# Autodesk Inventor assembly: Assembly
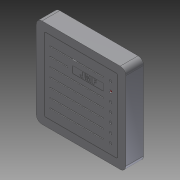
[picture p0: Inventor's stored thumbnail of the model, 180x180]
Saved by Autodesk Inventor 2012 (Build 160160000, 160)
## iProperties
Created: 2013-12-16
Part Number: Assembly
Document SubType Name: Assembly
Designer: joe_000
Author: joe_000
## Documents named in this file (5)
- C:\dev\stm32-rfid-clone\mechanical\Assembly.iam
- C:\dev\stm32-rfid-clone\mechanical\readerCase.ipt
- C:\dev\stm32-rfid-clone\mechanical\AABattery.ipt
- C:\dev\stm32-rfid-clone\mechanical\circuitBoard.ipt
- C:\dev\stm32-rfid-clone\mechanical\LED.ipt
## Components (7 placed, 4 different names)
1. readerCase:1 — Mate:5, Mate:6, Tangent:1, Tangent:2, Mate:7, Insert:1, Insert:2
2. AABattery:1 — Mate:2, Mate:3
3. AABattery:2 — Mate:1, Mate:4
4. AABattery:3 — Mate:2, Mate:3, Mate:6, Tangent:1
5. AABattery:4 — Mate:1, Mate:4, Mate:5, Tangent:2
6. circuitBoard:1 — Mate:7, Insert:1, Insert:2, Mate:8, Mate:9, Mate:10
7. LED:1 — Mate:8, Mate:9, Mate:10
## Relationships (14: Mate 10, Tangent 2, Insert 2)
- Mate:1: AABattery:2 ↔ AABattery:4
- Mate:2: AABattery:1 ↔ AABattery:3
- Mate:3: AABattery:1 ↔ AABattery:3
- Mate:4: AABattery:2 ↔ AABattery:4
- Mate:5: readerCase:1 ↔ AABattery:4
- Mate:6: readerCase:1 ↔ AABattery:3
- Tangent:1: readerCase:1 ↔ AABattery:3
- Tangent:2: readerCase:1 ↔ AABattery:4
- Mate:7: readerCase:1 ↔ circuitBoard:1
- Insert:1: readerCase:1 ↔ circuitBoard:1
- Insert:2: readerCase:1 ↔ circuitBoard:1
- Mate:8: circuitBoard:1 ↔ LED:1
- Mate:9: circuitBoard:1 ↔ LED:1
- Mate:10: circuitBoard:1 ↔ LED:1
